# Autodesk Inventor assembly: STEERING
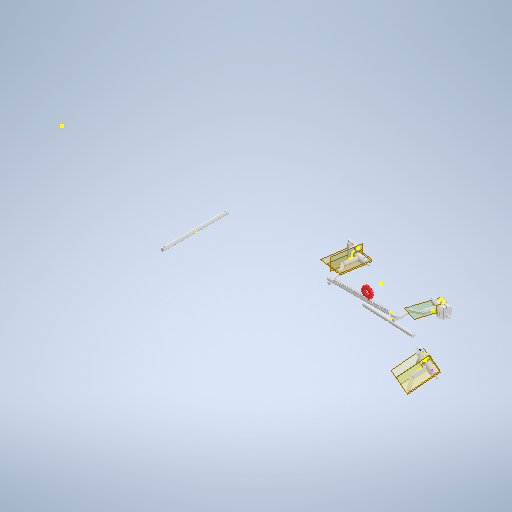
[picture p0: Inventor's stored thumbnail of the model, 512x512]
Saved by Autodesk Inventor 2025 (Build 290162010, 162A)
## iProperties
Created: 2024-08-11
Part Number: STEERING
Document SubType Name: Assembly
Designer: darkb
Author: darkb
## Documents named in this file (7)
- C:\Users\darkb\Desktop\newpartsBRANDNEW\STEERING.iam
- C:\Users\darkb\Desktop\newpartsBRANDNEW\TIE ROD.ipt
- C:\Users\darkb\Desktop\INVENTOR RC CAR\CONNETING CYLINDER.ipt
- C:\Users\darkb\Desktop\INVENTOR RC CAR\rack and pinion assembly.iam
- C:\Users\darkb\Desktop\newpartsBRANDNEW\SHAFT FOR STEERING 0.1 INCH.ipt
- C:\Users\darkb\Desktop\newpartsBRANDNEW\WHEEL ASSEMBLY.iam
- C:\Users\darkb\Desktop\newpartsBRANDNEW\WHEEL ASSEMBLY_MIR.iam
## Components (12 placed, 6 different names)
1. TIE ROD:1 — Mate:3, Mate:6
2. TIE ROD:2 — Mate:1, Mate:6
3. CONNETING CYLINDER:1
4. CONNETING CYLINDER:2
5. rack and pinion assembly:1 [sub-assembly] — Mate:1, Mate:3, Mate:5, Mate:7, Mate:8
6. SHAFT FOR STEERING 0.1 INCH:1 — Mate:7
7. SHAFT FOR STEERING 0.1 INCH:2 — Mate:8
8. SHAFT FOR STEERING 0.1 INCH:3 — Mate:9
9. SHAFT FOR STEERING 0.1 INCH:4 — Mate:10
10. WHEEL ASSEMBLY:1 [sub-assembly] — Mate:9
11. WHEEL ASSEMBLY:2 [sub-assembly]
12. WHEEL ASSEMBLY_MIR:1 [sub-assembly] — Mate:10
## Relationships (8: Mate 8)
- Mate:1: TIE ROD:2 ↔ rack and pinion assembly:1
- Mate:3: TIE ROD:1 ↔ rack and pinion assembly:1
- Mate:5: rack and pinion assembly:1
- Mate:6: TIE ROD:1 ↔ TIE ROD:2
- Mate:7: rack and pinion assembly:1 ↔ SHAFT FOR STEERING 0.1 INCH:1
- Mate:8: rack and pinion assembly:1 ↔ SHAFT FOR STEERING 0.1 INCH:2
- Mate:9: SHAFT FOR STEERING 0.1 INCH:3 ↔ WHEEL ASSEMBLY:1
- Mate:10: SHAFT FOR STEERING 0.1 INCH:4 ↔ WHEEL ASSEMBLY_MIR:1
